# Autodesk Inventor assembly: Mount_Mega
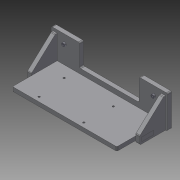
[picture p0: Inventor's stored thumbnail of the model, 180x180]
Saved by Autodesk Inventor 2014 (Build 180170000, 170)
## iProperties
Created: 2014-10-26
Part Number: Mount_Mega
Document SubType Name: Assembly
Designer: ThatOtherGuy
Author: ThatOtherGuy
## Documents named in this file (6)
- C:\Users\ThatOtherGuy\Documents\Inventor\KosselCNC1515\Mounts\Mount_Mega.iam
- C:\Users\ThatOtherGuy\Documents\Inventor\KosselCNC1515\Mounts\Mount_Mega_Back.ipt
- C:\Users\ThatOtherGuy\Documents\Inventor\KosselCNC1515\Mounts\Mount_Mega_Bottom.ipt
- C:\Users\ThatOtherGuy\Documents\Inventor\KosselCNC1515\Mounts\Mount_Mega_End.ipt
- C:\Users\ThatOtherGuy\Documents\Inventor\Content Center Files\R2014\en-US\DIN 562\DIN 562 - M3 x 5.5.ipt
- C:\Users\ThatOtherGuy\Documents\Inventor\Content Center Files\R2014\en-US\ANSI B18.3.1M(1)\ANSI B18.3.1M - M3x0.5 x 10(2).ipt
## Components (8 placed, 5 different names)
1. Mount_Mega_Bottom:1 — Mate:6, Mate:7, Mate:8, Mate:9, Mate:10, Mate:11, Mate:12
2. Mount_Mega_Back:1 — Mate:6, Mate:7, Mate:8, Mate:13, Mate:14, Insert:1, Insert:2, Insert:3, Insert:4
3. Mount_Mega_End:1 — Mate:11, Mate:12, Mate:14
4. Mount_Mega_End:2 — Mate:9, Mate:10, Mate:13
5. DIN 562 M3:1 — Insert:1
6. DIN 562 M3:2 — Insert:2
7. Broached Socket Head Cap Screw - Metric M3x0.5 x 10:1 — Insert:3
8. Broached Socket Head Cap Screw - Metric M3x0.5 x 10:2 — Insert:4
## Relationships (13: Mate 9, Insert 4)
- Mate:6: Mount_Mega_Bottom:1 ↔ Mount_Mega_Back:1
- Mate:7: Mount_Mega_Bottom:1 ↔ Mount_Mega_Back:1
- Mate:8: Mount_Mega_Bottom:1 ↔ Mount_Mega_Back:1
- Mate:9: Mount_Mega_Bottom:1 ↔ Mount_Mega_End:2
- Mate:10: Mount_Mega_Bottom:1 ↔ Mount_Mega_End:2
- Mate:11: Mount_Mega_Bottom:1 ↔ Mount_Mega_End:1
- Mate:12: Mount_Mega_Bottom:1 ↔ Mount_Mega_End:1
- Mate:13: Mount_Mega_Back:1 ↔ Mount_Mega_End:2
- Mate:14: Mount_Mega_Back:1 ↔ Mount_Mega_End:1
- Insert:1: Mount_Mega_Back:1 ↔ DIN 562 M3:1
- Insert:2: Mount_Mega_Back:1 ↔ DIN 562 M3:2
- Insert:3: Mount_Mega_Back:1 ↔ Broached Socket Head Cap Screw - Metric M3x0.5 x 10:1
- Insert:4: Mount_Mega_Back:1 ↔ Broached Socket Head Cap Screw - Metric M3x0.5 x 10:2
